# Autodesk Inventor assembly: motorized2
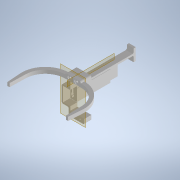
[picture p0: Inventor's stored thumbnail of the model, 180x180]
Saved by Autodesk Inventor 2020 (Build 240168000, 168)
## iProperties
Created: 2019-05-08
Part Number: motorized2
Document SubType Name: Assembly
Designer: erwin
Author: erwin
## Documents named in this file (5)
- D:\GitHub\ProtoSwitchBoard\design\pin-header_cutter\new_motorized\motorized2.iam
- D:\GitHub\ProtoSwitchBoard\design\pin-header_cutter\new_motorized\servo_bracket.ipt
- D:\GitHub\ProtoSwitchBoard\design\pin-header_cutter\new_motorized\leg.ipt
- D:\GitHub\ProtoSwitchBoard\design\pin-header_cutter\new_motorized\funnel.ipt
- D:\GitHub\ProtoSwitchBoard\design\pin-header_cutter\new_motorized\fence.ipt
## Components (4 placed, 4 different names)
1. servo_bracket:1 — Flush:1, Flush:2, Flush:3, Flush:4
2. leg:1 — Flush:1, Flush:2
3. funnel:1 — Flush:3
4. fence:1 — Flush:4
## Relationships (4: Flush 4)
- Flush:1: servo_bracket:1 ↔ leg:1
- Flush:2: servo_bracket:1 ↔ leg:1
- Flush:3: servo_bracket:1 ↔ funnel:1
- Flush:4: servo_bracket:1 ↔ fence:1
